# Autodesk Inventor assembly: BatteryCaseAssembly
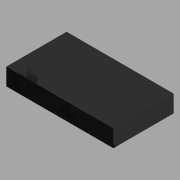
[picture p0: Inventor's stored thumbnail of the model, 180x180]
Saved by Autodesk Inventor 2017 (Build 210142000, 142)
## iProperties
Created: 2017-05-07
Part Number: BatteryCaseAssembly
Document SubType Name: Assembly
Designer: zallen
Author: zallen
## Documents named in this file (3)
- C:\Users\zallen\Documents\Autodesk Inventor Projects\LaundryRobot_v0.1\Base\Battery Pack Assembly\Battery Case Assembly\BatteryCaseAssembly.iam
- C:\Users\zallen\Documents\Autodesk Inventor Projects\LaundryRobot_v0.1\Base\Battery Pack Assembly\Battery Case Assembly\Battery Case Bottom.ipt
- C:\Users\zallen\Documents\Autodesk Inventor Projects\LaundryRobot_v0.1\Base\Battery Pack Assembly\Battery Case Assembly\Battery Case Top.ipt
## Components (2 placed, 2 different names)
1. Battery Case Bottom:1 — Mate:1, Mate:2
2. Battery Case Top:1 — Mate:1, Mate:2
## Relationships (2: Mate 2)
- Mate:1: Battery Case Bottom:1 ↔ Battery Case Top:1
- Mate:2: Battery Case Bottom:1 ↔ Battery Case Top:1
